# Autodesk Inventor assembly: Goal Capture
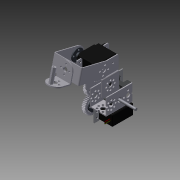
[picture p0: Inventor's stored thumbnail of the model, 180x180]
Saved by Autodesk Inventor 2014 SP2 (Build 180246200, 246)
## iProperties
Created: 2014-10-19
Part Number: Goal Capture
Document SubType Name: Assembly
Designer: Allison
Author: Allison
## Documents named in this file (18)
- C:\Users\Allison\Documents\inventor\InventorMasterProject\Goal Capture.iam
- C:\Users\Allison\Documents\Inventor\InventorMasterProject\Tetrix\Channel\32mm Channel.ipt
- C:\Users\Allison\Documents\Inventor\InventorMasterProject\Tetrix\Channel\96mm Channel.ipt
- C:\Users\Allison\Documents\Inventor\InventorMasterProject\Tetrix\Servos\Servo Assembly with horn.iam
- C:\Users\Allison\Documents\inventor\InventorMasterProject\Tetrix\Servos\Side Servo Mount.ipt
- C:\Users\Allison\Documents\Inventor\InventorMasterProject\Tetrix\Hubs and Axles\Bronze Bushing.ipt
- C:\Users\Allison\Documents\Inventor\InventorMasterProject\Tetrix\Hubs and Axles\Short Axle.ipt
- C:\Users\Allison\Documents\inventor\InventorMasterProject\Tetrix\Rack and Pinion\Pinion.ipt
- C:\Users\Allison\Documents\inventor\InventorMasterProject\Tetrix\Rack and Pinion\Slide Block.ipt
- C:\Users\Allison\Documents\Inventor\InventorMasterProject\Tetrix\Gears\40 Tooth Gear.ipt
- C:\Users\Allison\Documents\Inventor\InventorMasterProject\Tetrix\Hubs and Axles\Axle Hub.ipt
- C:\Users\Allison\Documents\inventor\InventorMasterProject\Tetrix\Servos\Servo Mount.ipt
- C:\Users\Allison\Documents\inventor\InventorMasterProject\Tetrix\Servos\Servo Pivot Bracket.ipt
- C:\Users\Allison\Documents\inventor\InventorMasterProject\Tetrix\Brackets\L-Bracket.ipt
- C:\Users\Allison\Documents\inventor\InventorMasterProject\Tetrix\Standoffs\1 Inch Standoff.ipt
- C:\Users\Allison\Documents\Inventor\InventorMasterProject\Tetrix\Servos\Servo.ipt
- C:\Users\Allison\Documents\Inventor\InventorMasterProject\Tetrix\Servos\Servo Horn Metal.ipt
- C:\Users\Allison\Documents\Inventor\InventorMasterProject\Tetrix\Spacers\Nylon Spacer 0.125in.ipt
## Components (19 placed, 17 different names)
1. 32mm Channel:1 — Flush:1, Mate:3, Insert:12, Insert:13
2. 96mm Channel:1 — Insert:1, Mate:1, Insert:3, Insert:6
3. Servo Assembly with horn:1 [sub-assembly] — Insert:2, Insert:5
4. Bronze Bushing:1 — Insert:6, Insert:7
5. Short Axle:1 — Mate:1, Mate:2
6. Pinion:1 — Mate:2
7. Slide Block:1 — Insert:3
8. Side Servo Mount:2 — Insert:1, Insert:2, Flush:1, Mate:3
9. 40 Tooth Gear:1 — Insert:4
10. 40 Tooth Gear:2 — Insert:5
11. Axle Hub:1 — Insert:4, Insert:7
12. Servo:1 — Insert:17, Insert:18, Insert:19
13. Servo Mount:1 — Insert:12, Insert:13, Insert:17, Insert:18, Insert:24, Insert:25
14. Servo Pivot Bracket:1 — Insert:20, Insert:21, Insert:22, Insert:23
15. L-Bracket:1 — Insert:16, Insert:22, Insert:23
16. 1 Inch Standoff:1 — Insert:16
17. Servo Horn Metal:1 — Insert:19, Insert:20, Insert:21
18. Nylon Spacer 0.125in:1 — Insert:24
19. Nylon Spacer 0.125in:2 — Insert:25
## Relationships (23: Insert 19, Mate 3, Flush 1)
- Insert:1: 96mm Channel:1 ↔ Side Servo Mount:2
- Insert:2: Servo Assembly with horn:1 ↔ Side Servo Mount:2
- Mate:1: 96mm Channel:1 ↔ Short Axle:1
- Mate:2: Short Axle:1 ↔ Pinion:1
- Insert:3: 96mm Channel:1 ↔ Slide Block:1
- Insert:4: 40 Tooth Gear:1 ↔ Axle Hub:1
- Insert:5: Servo Assembly with horn:1 ↔ 40 Tooth Gear:2
- Insert:6: 96mm Channel:1 ↔ Bronze Bushing:1
- Insert:7: Bronze Bushing:1 ↔ Axle Hub:1
- Flush:1: 32mm Channel:1 ↔ Side Servo Mount:2
- Mate:3: 32mm Channel:1 ↔ Side Servo Mount:2
- Insert:12 (3.175 mm): 32mm Channel:1 ↔ Servo Mount:1
- Insert:13 (3.175 mm): 32mm Channel:1 ↔ Servo Mount:1
- Insert:16: L-Bracket:1 ↔ 1 Inch Standoff:1
- Insert:17: Servo:1 ↔ Servo Mount:1
- Insert:18: Servo:1 ↔ Servo Mount:1
- Insert:19: Servo:1 ↔ Servo Horn Metal:1
- Insert:20: Servo Pivot Bracket:1 ↔ Servo Horn Metal:1
- Insert:21: Servo Pivot Bracket:1 ↔ Servo Horn Metal:1
- Insert:22: Servo Pivot Bracket:1 ↔ L-Bracket:1
- Insert:23: Servo Pivot Bracket:1 ↔ L-Bracket:1
- Insert:24: Servo Mount:1 ↔ Nylon Spacer 0.125in:1
- Insert:25: Servo Mount:1 ↔ Nylon Spacer 0.125in:2
